# Autodesk Inventor assembly: CanSat
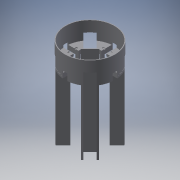
[picture p0: Inventor's stored thumbnail of the model, 180x180]
Saved by Autodesk Inventor 2018 (Build 220112000, 112)
## iProperties
Created: 2018-05-01
Part Number: CanSat
Document SubType Name: Assembly
Designer: suchanek
Author: suchanek
## Documents named in this file (6)
- C:\Users\sucha\programming\CanSat\CanSat2.0\Schematics\Model\CanSat.iam
- C:\Users\sucha\programming\CanSat\CanSat2.0\Schematics\Model\Hull_middle.ipt
- C:\Users\sucha\programming\CanSat\CanSat2.0\Schematics\Model\Hull_batt_pillar.ipt
- C:\Users\sucha\programming\CanSat\CanSat2.0\Schematics\Model\Circuit.ipt
- C:\Users\sucha\programming\CanSat\CanSat2.0\Schematics\Model\Motor_drivers.ipt
- C:\Users\sucha\programming\CanSat\CanSat2.0\Schematics\Model\Hull_main.ipt
## Components (8 placed, 5 different names)
1. Hull_middle:1 — Rotational:2, Angle:2, Rotational:3
2. Circuit:1 — Rotational:2, Angle:2, Angle:3
3. Motor_drivers:1 — Flush:1, Angle:4, Cylindrical:1
4. Hull_main:1 — Rotational:1, Angle:1, Rotational:3, Angle:3, Flush:1, Angle:4, Cylindrical:1
5. Hull_batt_pillar:1 — Rotational:1, Angle:1
6. Hull_batt_pillar:2
7. Hull_batt_pillar:3
8. Hull_batt_pillar:4
## Component patterns: (4 elements, first: Hull_batt_pillar:1)
## Relationships (9: Angle 4, RevoluteJoint 3, Flush 1, CylindricalJoint 1)
- Rotational:1 [RevoluteJoint]: Hull_main:1 ↔ Hull_batt_pillar:1
- Angle:1 (0 deg): Hull_main:1 ↔ Hull_batt_pillar:1
- Rotational:2 [RevoluteJoint]: Hull_middle:1 ↔ Circuit:1
- Angle:2 (0 deg): Hull_middle:1 ↔ Circuit:1
- Rotational:3 [RevoluteJoint]: Hull_middle:1 ↔ Hull_main:1
- Angle:3 (0 deg): Circuit:1 ↔ Hull_main:1
- Flush:1 (12 mm): Motor_drivers:1 ↔ Hull_main:1
- Angle:4 (0 deg): Motor_drivers:1 ↔ Hull_main:1
- Cylindrical:1: Motor_drivers:1 ↔ Hull_main:1
